# Autodesk Inventor assembly: Assembly2
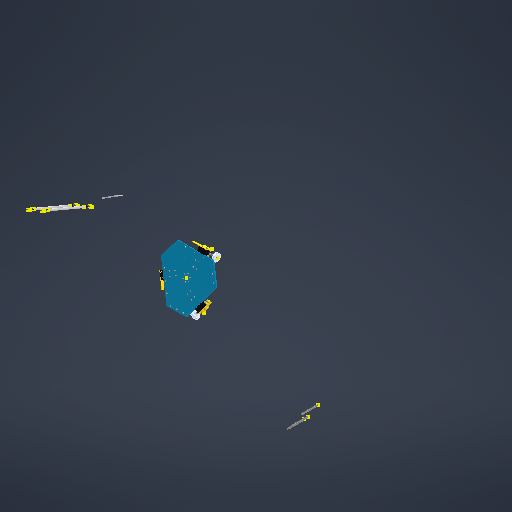
[picture p0: Inventor's stored thumbnail of the model, 512x512]
Saved by Autodesk Inventor 2027.1 (Build 311270010, 270A)
## iProperties
Created: 2026-08-09
Part Number: Assembly2
Document SubType Name: Assembly
Designer: MSI
Author: MSI
## Documents named in this file (19)
- C:\Users\MSI\Documents\MECHATRONICS\Tot_nghiep\Do_an_Delta.Robot_Dang_Rui_Bi\Thiết kế\Delta Part\Assembly2.iam
- C:\Users\MSI\Documents\MECHATRONICS\Tot_nghiep\Do_an_Delta.Robot_Dang_Rui_Bi\Thiết kế\Delta Part\đế trên.ipt
- C:\Users\MSI\Documents\Inventor\Content Center Files\R2027\en-US\AS 1427(08)\AS 1427 - M4 x 6(6) I.ipt
- C:\Users\MSI\Documents\MECHATRONICS\Tot_nghiep\Do_an_Delta.Robot_Dang_Rui_Bi\Thiết kế\Delta Part\nhôm định hình đôi_gá link1.ipt
- C:\Users\MSI\Documents\MECHATRONICS\Tot_nghiep\Do_an_Delta.Robot_Dang_Rui_Bi\Thiết kế\Delta Part\Hộp trượt vòng bi.ipt
- C:\Users\MSI\Documents\MECHATRONICS\Tot_nghiep\Do_an_Delta.Robot_Dang_Rui_Bi\Thiết kế\Tool_STL\Part1.ipt
- C:\Users\MSI\Documents\Inventor\Content Center Files\R2027\en-US\AS 1427(08)\AS 1427 - M4 x 12(6) I.ipt
- C:\Users\MSI\Documents\Inventor\Content Center Files\R2027\en-US\AS 1427(08)\AS 1427 - M4 x 25(6) I.ipt
- C:\Users\MSI\Documents\Inventor\Content Center Files\R2027\en-US\BS 3692(1)\BS 3692 - M4(1).ipt
- C:\Users\MSI\Documents\MECHATRONICS\Tot_nghiep\Do_an_Delta.Robot_Dang_Rui_Bi\Thiết kế\Delta Part\trục đai.ipt
- C:\Users\MSI\Documents\MECHATRONICS\Tot_nghiep\Do_an_Delta.Robot_Dang_Rui_Bi\Thiết kế\Delta Part\GT2_60.ipt
- C:\Users\MSI\Documents\MECHATRONICS\Tot_nghiep\Do_an_Delta.Robot_Dang_Rui_Bi\Thiết kế\Delta Part\khóa trục.ipt
- C:\Users\MSI\Documents\MECHATRONICS\Tot_nghiep\Do_an_Delta.Robot_Dang_Rui_Bi\Thiết kế\Delta Part\mặt bích.ipt
- C:\Users\MSI\Documents\Inventor\Content Center Files\R2027\en-US\BS EN ISO 4026\BS EN ISO 4168 - M3 x 3(2).ipt
- C:\Users\MSI\Documents\Inventor\Content Center Files\R2027\en-US\AS 1427(05)\AS 1427 - M2.5 x 4(5) II.ipt
- C:\Users\MSI\Documents\MECHATRONICS\Tot_nghiep\Do_an_Delta.Robot_Dang_Rui_Bi\Thiết kế\Delta Part\Link1.ipt
- C:\Users\MSI\Documents\MECHATRONICS\Tot_nghiep\Do_an_Delta.Robot_Dang_Rui_Bi\Thiết kế\Delta Part\khớp nối mắt trâu lỗ 4mm.iam
- C:\Users\MSI\Documents\MECHATRONICS\Tot_nghiep\Do_an_Delta.Robot_Dang_Rui_Bi\Thiết kế\Delta Part\link2.ipt
- C:\Users\MSI\Documents\MECHATRONICS\Tot_nghiep\Do_an_Delta.Robot_Dang_Rui_Bi\Thiết kế\Delta Part\khớp nối.ipt
## Components (104 placed, 18 different names)
1. đế trên:1 — Insert:1, Insert:2, Insert:3, Insert:4, Insert:5, Insert:6, Insert:7, Insert:8, Insert:9, Insert:10, Insert:11, Insert:12, Insert:13, Insert:14, Insert:15, Insert:16, Insert:17, Insert:18, Mate:1, Mate:2, Mate:3, Mate:4, Mate:5, Mate:6, Mate:7, Mate:8, Mate:9, Insert:27, Insert:28, Insert:29, Insert:30, Insert:31, Insert:32, Insert:33, Insert:34, Insert:35, Insert:36, Insert:37, Insert:38, Insert:39, Insert:40, Insert:41, Insert:42, Insert:43, Insert:44, Insert:45, Insert:46, Insert:47, Insert:52, Insert:55, Insert:56, Insert:57, Insert:58, Insert:59, Insert:60, Insert:61, Insert:62
2. AS 1427 Z - Metric M4 x 12:3 — Insert:1
3. AS 1427 Z - Metric M4 x 12:4 — Insert:2
4. AS 1427 Z - Metric M4 x 12:5 — Insert:3
5. AS 1427 Z - Metric M4 x 12:6 — Insert:4
6. AS 1427 Z - Metric M4 x 12:7 — Insert:5
7. AS 1427 Z - Metric M4 x 12:8 — Insert:6
8. AS 1427 Z - Metric M4 x 12:9 — Insert:7
9. AS 1427 Z - Metric M4 x 12:10 — Insert:8
10. AS 1427 Z - Metric M4 x 12:11 — Insert:9
11. AS 1427 Z - Metric M4 x 12:12 — Insert:10
12. AS 1427 Z - Metric M4 x 12:13 — Insert:11
13. AS 1427 Z - Metric M4 x 12:14 — Insert:12
14. AS 1427 Z - Metric M4 x 12:15 — Insert:13
15. AS 1427 Z - Metric M4 x 12:16 — Insert:14
16. AS 1427 Z - Metric M4 x 12:17 — Insert:15
17. AS 1427 Z - Metric M4 x 12:18 — Insert:16
18. AS 1427 Z - Metric M4 x 12:19 — Insert:17
19. AS 1427 Z - Metric M4 x 12:20 — Insert:18
20. nhôm định hình đôi_gá link1:1 — Mate:1, Mate:2, Mate:3, Mate:14, Flush:3, Mate:15, Mate:17, Flush:6, Flush:7, Insert:63, Insert:64, Insert:65, Insert:66
21. nhôm định hình đôi_gá link1:2 — Mate:4, Mate:5, Mate:6, Mate:12, Flush:2, Mate:13, Mate:18, Flush:8, Flush:9, Insert:48, Insert:49, Insert:50, Insert:51
22. nhôm định hình đôi_gá link1:3 — Mate:7, Mate:8, Mate:9, Mate:10, Flush:1, Mate:11, Flush:4, Flush:5, Insert:67, Insert:68, Insert:69, Insert:70
23. Hộp trượt vòng bi:1 — Mate:10, Flush:1, Mate:11, Mate:16, Mate:30
24. Hộp trượt vòng bi:2 — Mate:14, Flush:3, Mate:15, Mate:23, Mate:24, Mate:26
25. Hộp trượt vòng bi:3 — Mate:12, Flush:2, Mate:13, Mate:21, Mate:22, Mate:28
26. Part1:1 — Mate:17, Flush:6, Flush:7, Insert:75, Insert:76
27. Part1:2 — Mate:18, Flush:8, Flush:9, Insert:73, Insert:74
28. Part1:3 — Mate:16, Flush:4, Flush:5, Insert:71, Insert:72
29. AS 1427 Z - Metric M4 x 25:2 — Insert:27
30. AS 1427 Z - Metric M4 x 25:3 — Insert:28
31. AS 1427 Z - Metric M4 x 25:4 — Insert:29
32. AS 1427 Z - Metric M4 x 25:5 — Insert:30
33. BS 3692 - Metric M4:1 — Insert:31
34. BS 3692 - Metric M4:2 — Insert:32
35. BS 3692 - Metric M4:3 — Insert:33
36. BS 3692 - Metric M4:4 — Insert:34
37. BS 3692 - Metric M4:5 — Insert:35
38. BS 3692 - Metric M4:6 — Insert:36
39. BS 3692 - Metric M4:7 — Insert:37
40. BS 3692 - Metric M4:8 — Insert:38
41. BS 3692 - Metric M4:9 — Insert:39
42. BS 3692 - Metric M4:10 — Insert:40
43. BS 3692 - Metric M4:11 — Insert:41
44. BS 3692 - Metric M4:12 — Insert:42
45. BS 3692 - Metric M4:13 — Insert:43
46. BS 3692 - Metric M4:14 — Insert:44
47. BS 3692 - Metric M4:15 — Insert:45
48. BS 3692 - Metric M4:16 — Insert:46
49. BS 3692 - Metric M4:17 — Insert:47
50. BS 3692 - Metric M4:18 — Insert:48
51. BS 3692 - Metric M4:19 — Insert:49
52. BS 3692 - Metric M4:20 — Insert:50
53. BS 3692 - Metric M4:21 — Insert:51
54. BS 3692 - Metric M4:22 — Insert:52
55. AS 1427 Z - Metric M4 x 25:8 — Insert:55
56. AS 1427 Z - Metric M4 x 25:9 — Insert:56
57. AS 1427 Z - Metric M4 x 25:10 — Insert:57
58. AS 1427 Z - Metric M4 x 25:11 — Insert:58
59. AS 1427 Z - Metric M4 x 25:12 — Insert:59
60. AS 1427 Z - Metric M4 x 25:13 — Insert:60
61. AS 1427 Z - Metric M4 x 25:14 — Insert:61
62. AS 1427 Z - Metric M4 x 25:15 — Insert:62
63. BS 3692 - Metric M4:23 — Insert:63
64. BS 3692 - Metric M4:24 — Insert:64
65. BS 3692 - Metric M4:25 — Insert:65
66. BS 3692 - Metric M4:26 — Insert:66
67. BS 3692 - Metric M4:27 — Insert:67
68. BS 3692 - Metric M4:28 — Insert:68
69. BS 3692 - Metric M4:29 — Insert:69
70. BS 3692 - Metric M4:30 — Insert:70
71. AS 1427 Z - Metric M4 x 6:1 — Insert:71
72. AS 1427 Z - Metric M4 x 6:2 — Insert:72
73. AS 1427 Z - Metric M4 x 6:3 — Insert:73
74. AS 1427 Z - Metric M4 x 6:4 — Insert:74
75. AS 1427 Z - Metric M4 x 6:5 — Insert:75
76. AS 1427 Z - Metric M4 x 6:6 — Insert:76
77. trục đai:2 — Mate:23, Mate:24, Mate:25, Mate:33, Flush:12, Mate:38, Mate:39, Mate:43
78. trục đai:3 — Mate:21, Mate:22, Mate:27, Mate:31, Flush:10, Mate:36, Mate:37
79. GT2_60:1
80. GT2_60:2 — Mate:33, Flush:12
81. GT2_60:3 — Mate:31, Flush:10
82. khóa trục:1 — Mate:25, Mate:26
83. khóa trục:2 — Mate:30
84. khóa trục:3 — Mate:27, Mate:28
85. mặt bích:1 — Mate:36, Mate:37, Mate:44
86. mặt bích:3 — Mate:40
87. mặt bích:4 — Mate:38, Mate:39, Mate:41, Mate:42
88. BS EN ISO 4026 - Metric M3 x 3:1 — Mate:40
89. AS 1427 H - Metric M2.5 x 4:1 — Mate:41, Mate:42, Mate:43
90. AS 1427 H - Metric M2.5 x 4:2 — Mate:44
91. khớp nối mắt trâu lỗ 4mm:15 [sub-assembly]
92. khớp nối mắt trâu lỗ 4mm:16 [sub-assembly]
93. link2:8
94. khớp nối:15
95. khớp nối:16
96. khớp nối mắt trâu lỗ 4mm:17 [sub-assembly]
97. khớp nối mắt trâu lỗ 4mm:18 [sub-assembly]
98. link2:9
99. khớp nối:17
100. khớp nối:18
101. Link1:4
102. trục đai:4
103. trục đai:5
104. trục đai:6
## Relationships (135: Insert 66, Mate 56, Flush 13)
- Insert:1: đế trên:1 ↔ AS 1427 Z - Metric M4 x 12:3
- Insert:2: đế trên:1 ↔ AS 1427 Z - Metric M4 x 12:4
- Insert:3: đế trên:1 ↔ AS 1427 Z - Metric M4 x 12:5
- Insert:4: đế trên:1 ↔ AS 1427 Z - Metric M4 x 12:6
- Insert:5: đế trên:1 ↔ AS 1427 Z - Metric M4 x 12:7
- Insert:6: đế trên:1 ↔ AS 1427 Z - Metric M4 x 12:8
- Insert:7: đế trên:1 ↔ AS 1427 Z - Metric M4 x 12:9
- Insert:8: đế trên:1 ↔ AS 1427 Z - Metric M4 x 12:10
- Insert:9: đế trên:1 ↔ AS 1427 Z - Metric M4 x 12:11
- Insert:10: đế trên:1 ↔ AS 1427 Z - Metric M4 x 12:12
- Insert:11: đế trên:1 ↔ AS 1427 Z - Metric M4 x 12:13
- Insert:12: đế trên:1 ↔ AS 1427 Z - Metric M4 x 12:14
- Insert:13: đế trên:1 ↔ AS 1427 Z - Metric M4 x 12:15
- Insert:14: đế trên:1 ↔ AS 1427 Z - Metric M4 x 12:16
- Insert:15: đế trên:1 ↔ AS 1427 Z - Metric M4 x 12:17
- Insert:16: đế trên:1 ↔ AS 1427 Z - Metric M4 x 12:18
- Insert:17: đế trên:1 ↔ AS 1427 Z - Metric M4 x 12:19
- Insert:18: đế trên:1 ↔ AS 1427 Z - Metric M4 x 12:20
- Mate:1: đế trên:1 ↔ nhôm định hình đôi_gá link1:1
- Mate:2: đế trên:1 ↔ nhôm định hình đôi_gá link1:1
- Mate:3: đế trên:1 ↔ nhôm định hình đôi_gá link1:1
- Mate:4: đế trên:1 ↔ nhôm định hình đôi_gá link1:2
- Mate:5: đế trên:1 ↔ nhôm định hình đôi_gá link1:2
- Mate:6: đế trên:1 ↔ nhôm định hình đôi_gá link1:2
- Mate:7: đế trên:1 ↔ nhôm định hình đôi_gá link1:3
- Mate:8: đế trên:1 ↔ nhôm định hình đôi_gá link1:3
- Mate:9: đế trên:1 ↔ nhôm định hình đôi_gá link1:3
- Mate:10: nhôm định hình đôi_gá link1:3 ↔ Hộp trượt vòng bi:1
- Flush:1: nhôm định hình đôi_gá link1:3 ↔ Hộp trượt vòng bi:1
- Mate:11: nhôm định hình đôi_gá link1:3 ↔ Hộp trượt vòng bi:1
- Mate:12: nhôm định hình đôi_gá link1:2 ↔ Hộp trượt vòng bi:3
- Flush:2: nhôm định hình đôi_gá link1:2 ↔ Hộp trượt vòng bi:3
- Mate:13: nhôm định hình đôi_gá link1:2 ↔ Hộp trượt vòng bi:3
- Mate:14: nhôm định hình đôi_gá link1:1 ↔ Hộp trượt vòng bi:2
- Flush:3: nhôm định hình đôi_gá link1:1 ↔ Hộp trượt vòng bi:2
- Mate:15: nhôm định hình đôi_gá link1:1 ↔ Hộp trượt vòng bi:2
- Mate:16: Hộp trượt vòng bi:1 ↔ Part1:3
- Flush:4: nhôm định hình đôi_gá link1:3 ↔ Part1:3
- Flush:5: nhôm định hình đôi_gá link1:3 ↔ Part1:3
- Mate:17: nhôm định hình đôi_gá link1:1 ↔ Part1:1
- Flush:6: nhôm định hình đôi_gá link1:1 ↔ Part1:1
- Flush:7: nhôm định hình đôi_gá link1:1 ↔ Part1:1
- Mate:18: nhôm định hình đôi_gá link1:2 ↔ Part1:2
- Flush:8: nhôm định hình đôi_gá link1:2 ↔ Part1:2
- Flush:9: nhôm định hình đôi_gá link1:2 ↔ Part1:2
- Insert:27: đế trên:1 ↔ AS 1427 Z - Metric M4 x 25:2
- Insert:28: đế trên:1 ↔ AS 1427 Z - Metric M4 x 25:3
- Insert:29: đế trên:1 ↔ AS 1427 Z - Metric M4 x 25:4
- Insert:30: đế trên:1 ↔ AS 1427 Z - Metric M4 x 25:5
- Insert:31: đế trên:1 ↔ BS 3692 - Metric M4:1
- Insert:32: đế trên:1 ↔ BS 3692 - Metric M4:2
- Insert:33: đế trên:1 ↔ BS 3692 - Metric M4:3
- Insert:34: đế trên:1 ↔ BS 3692 - Metric M4:4
- Insert:35: đế trên:1 ↔ BS 3692 - Metric M4:5
- Insert:36: đế trên:1 ↔ BS 3692 - Metric M4:6
- Insert:37: đế trên:1 ↔ BS 3692 - Metric M4:7
- Insert:38: đế trên:1 ↔ BS 3692 - Metric M4:8
- Insert:39: đế trên:1 ↔ BS 3692 - Metric M4:9
- Insert:40: đế trên:1 ↔ BS 3692 - Metric M4:10
- Insert:41: đế trên:1 ↔ BS 3692 - Metric M4:11
- Insert:42: đế trên:1 ↔ BS 3692 - Metric M4:12
- Insert:43: đế trên:1 ↔ BS 3692 - Metric M4:13
- Insert:44: đế trên:1 ↔ BS 3692 - Metric M4:14
- Insert:45: đế trên:1 ↔ BS 3692 - Metric M4:15
- Insert:46: đế trên:1 ↔ BS 3692 - Metric M4:16
- Insert:47: đế trên:1 ↔ BS 3692 - Metric M4:17
- Insert:48: nhôm định hình đôi_gá link1:2 ↔ BS 3692 - Metric M4:18
- Insert:49: nhôm định hình đôi_gá link1:2 ↔ BS 3692 - Metric M4:19
- Insert:50: nhôm định hình đôi_gá link1:2 ↔ BS 3692 - Metric M4:20
- Insert:51: nhôm định hình đôi_gá link1:2 ↔ BS 3692 - Metric M4:21
- Insert:52: đế trên:1 ↔ BS 3692 - Metric M4:22
- Insert:55: đế trên:1 ↔ AS 1427 Z - Metric M4 x 25:8
- Insert:56: đế trên:1 ↔ AS 1427 Z - Metric M4 x 25:9
- Insert:57: đế trên:1 ↔ AS 1427 Z - Metric M4 x 25:10
- Insert:58: đế trên:1 ↔ AS 1427 Z - Metric M4 x 25:11
- Insert:59: đế trên:1 ↔ AS 1427 Z - Metric M4 x 25:12
- Insert:60: đế trên:1 ↔ AS 1427 Z - Metric M4 x 25:13
- Insert:61: đế trên:1 ↔ AS 1427 Z - Metric M4 x 25:14
- Insert:62: đế trên:1 ↔ AS 1427 Z - Metric M4 x 25:15
- Insert:63: nhôm định hình đôi_gá link1:1 ↔ BS 3692 - Metric M4:23
- Insert:64: nhôm định hình đôi_gá link1:1 ↔ BS 3692 - Metric M4:24
- Insert:65: nhôm định hình đôi_gá link1:1 ↔ BS 3692 - Metric M4:25
- Insert:66: nhôm định hình đôi_gá link1:1 ↔ BS 3692 - Metric M4:26
- Insert:67: nhôm định hình đôi_gá link1:3 ↔ BS 3692 - Metric M4:27
- Insert:68: nhôm định hình đôi_gá link1:3 ↔ BS 3692 - Metric M4:28
- Insert:69: nhôm định hình đôi_gá link1:3 ↔ BS 3692 - Metric M4:29
- Insert:70: nhôm định hình đôi_gá link1:3 ↔ BS 3692 - Metric M4:30
- Insert:71: Part1:3 ↔ AS 1427 Z - Metric M4 x 6:1
- Insert:72: Part1:3 ↔ AS 1427 Z - Metric M4 x 6:2
- Insert:73: Part1:2 ↔ AS 1427 Z - Metric M4 x 6:3
- Insert:74: Part1:2 ↔ AS 1427 Z - Metric M4 x 6:4
- Insert:75: Part1:1 ↔ AS 1427 Z - Metric M4 x 6:5
- Insert:76: Part1:1 ↔ AS 1427 Z - Metric M4 x 6:6
- Mate:21: Hộp trượt vòng bi:3 ↔ trục đai:3
- Mate:22: Hộp trượt vòng bi:3 ↔ trục đai:3
- Mate:23: Hộp trượt vòng bi:2 ↔ trục đai:2
- Mate:24: Hộp trượt vòng bi:2 ↔ trục đai:2
- Mate:25: trục đai:2 ↔ khóa trục:1
- Mate:26: Hộp trượt vòng bi:2 ↔ khóa trục:1
- Mate:27: trục đai:3 ↔ khóa trục:3
- Mate:28: Hộp trượt vòng bi:3 ↔ khóa trục:3
- Mate:30: Hộp trượt vòng bi:1 ↔ khóa trục:2
- Mate:31: trục đai:3 ↔ GT2_60:3
- Flush:10: trục đai:3 ↔ GT2_60:3
- Mate:33: trục đai:2 ↔ GT2_60:2
- Flush:12: trục đai:2 ↔ GT2_60:2
- Mate:36: trục đai:3 ↔ mặt bích:1
- Mate:37: trục đai:3 ↔ mặt bích:1
- Mate:38: trục đai:2 ↔ mặt bích:4
- Mate:39: trục đai:2 ↔ mặt bích:4
- Mate:40: mặt bích:3 ↔ BS EN ISO 4026 - Metric M3 x 3:1
- Mate:41: mặt bích:4 ↔ AS 1427 H - Metric M2.5 x 4:1
- Mate:42: mặt bích:4 ↔ AS 1427 H - Metric M2.5 x 4:1
- Mate:43: trục đai:2 ↔ AS 1427 H - Metric M2.5 x 4:1
- Mate:44: mặt bích:1 ↔ AS 1427 H - Metric M2.5 x 4:2
- [Mate]: khớp nối mắt trâu lỗ 4mm:16 ↔ khớp nối:16
- [Mate]: khớp nối mắt trâu lỗ 4mm:16 ↔ khớp nối:16
- [Mate]: link2:8 ↔ khớp nối:16
- [Mate]: link2:8 ↔ khớp nối:16
- [Mate]: link2:8 ↔ khớp nối:15
- [Mate]: khớp nối mắt trâu lỗ 4mm:15 ↔ khớp nối:15
- [Mate]: khớp nối mắt trâu lỗ 4mm:15 ↔ khớp nối:15
- [Mate]: khớp nối mắt trâu lỗ 4mm:15 ↔ khớp nối:15
- [Mate]: link2:8 ↔ khớp nối:15
- [Flush]: khớp nối mắt trâu lỗ 4mm:15 ↔ khớp nối mắt trâu lỗ 4mm:16
- [Mate]: khớp nối mắt trâu lỗ 4mm:18 ↔ khớp nối:18
- [Mate]: khớp nối mắt trâu lỗ 4mm:18 ↔ khớp nối:18
- [Mate]: link2:9 ↔ khớp nối:18
- [Mate]: link2:9 ↔ khớp nối:18
- [Mate]: link2:9 ↔ khớp nối:17
- [Mate]: khớp nối mắt trâu lỗ 4mm:17 ↔ khớp nối:17
- [Mate]: khớp nối mắt trâu lỗ 4mm:17 ↔ khớp nối:17
- [Mate]: khớp nối mắt trâu lỗ 4mm:17 ↔ khớp nối:17
- [Mate]: link2:9 ↔ khớp nối:17
- [Flush]: khớp nối mắt trâu lỗ 4mm:17 ↔ khớp nối mắt trâu lỗ 4mm:18
## Named parameters: d407_d383 = 0 mm, d408_d384 = 0 mm, d409_d390 = 0 mm, d410_d358_d323 = 0 mm, d411_d359_d324 = 0 mm, d412_d360_d325 = 0 mm, d413_d361_d326 = 0 mm, d414_d362_d327 = 0 mm, d415_d363_d328 = 0 mm, d416_d364_d329 = 0 mm, d417_d383 = 0 mm, d418_d384 = 0 mm, d419_d390 = 0 mm, d420_d358_d323 = 0 mm, d421_d359_d324 = 0 mm, d422_d360_d325 = 0 mm, d423_d361_d326 = 0 mm, d424_d362_d327 = 0 mm, d425_d363_d328 = 0 mm, d426_d364_d329 = 0 mm
